# Autodesk Inventor assembly: kinect_ring_back
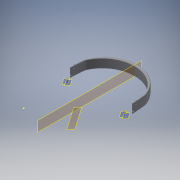
[picture p0: Inventor's stored thumbnail of the model, 180x180]
Saved by Autodesk Inventor 2019 (Build 230136000, 136)
## iProperties
Created: 2024-05-03
Part Number: kinect_ring_back
Material: Generisch
Document SubType Name: Assembly
Designer: nic
Author: nic
## Documents named in this file (2)
- C:\Users\Nicolas Frick\Sync\OneDrive\wtm\nicol_rh8d\atxmega_qenc\inventor\kinect_ring_back.iam
- C:\Users\Nicolas Frick\Sync\OneDrive\wtm\nicol_rh8d\atxmega_qenc\inventor\kinect_ring_back.ipt
## Components (1 placed, 1 different names)
1. kinect_ring_back:1 — Passend:1
## Relationships (1: Mate 1)
- Passend:1 [Mate]: kinect_ring_back:1
